# Autodesk Inventor assembly: derive_baseplate_v15
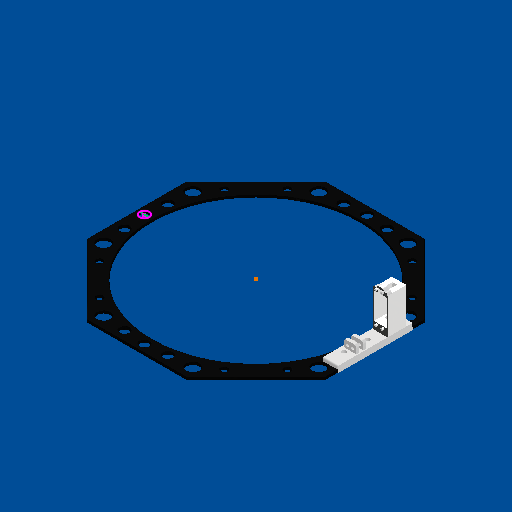
[picture p0: Inventor's stored thumbnail of the model, 512x512]
Saved by Autodesk Inventor 2026.2 (Build 302298000, 298)
## iProperties
Created: 2026-02-19
Part Number: derive_baseplate_v15
Document SubType Name: Assembly
Designer: Thoma
Author: Thoma
## Documents named in this file (3)
- C:\Users\Thoma\OneDrive\Desktop\dir\telescope_cover\cover\derive_baseplate_v15.iam
- C:\Users\Thoma\OneDrive\Desktop\dir\telescope_cover\telescope\version_4\Telescope_End.ipt
- C:\Users\Thoma\OneDrive\Desktop\dir\telescope_cover\cover\base_plate_v14.ipt
## Components (2 placed, 2 different names)
1. Telescope_End:1 — Flush:1, Angle:1, Mate:1
2. base_plate_v14:1 — Flush:1, Angle:1, Mate:1
## Relationships (3: Flush 1, Angle 1, Mate 1)
- Flush:1: Telescope_End:1 ↔ base_plate_v14:1
- Angle:1 (0 deg): Telescope_End:1 ↔ base_plate_v14:1
- Mate:1: Telescope_End:1 ↔ base_plate_v14:1
